# Autodesk Inventor assembly: BracoRobotico_FINAL_9999_999
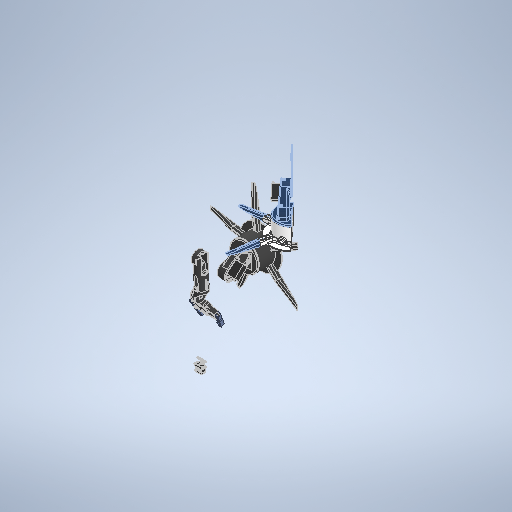
[picture p0: Inventor's stored thumbnail of the model, 512x512]
Saved by Autodesk Inventor 2025.2 (Build 292293000, 293)
## iProperties
Created: 2025-06-01
Part Number: BracoRobotico_FINAL_9999_999
Document SubType Name: Assembly
Designer: Gustavo Sousa
Author: Gustavo Sousa
## Documents named in this file (19)
- C:\Users\lucas\OneDrive\Documentos\Documentos\Gustavo\Mozangao\Projeto Base (5140)\correcao_pecas_braco_robotico\Braço Robotico peças corrigidas\BracoRobotico_FINAL_9999_999.iam
- C:\Users\lucas\OneDrive\Documentos\Documentos\Gustavo\Mozangao\Projeto Base (5140)\correcao_pecas_braco_robotico\Braço Robotico peças corrigidas\BracoRobotico_0004_001.ipt
- C:\Users\lucas\OneDrive\Documentos\Documentos\Gustavo\Mozangao\Projeto Base (5140)\correcao_pecas_braco_robotico\Braço Robotico peças corrigidas\BracoRobotico_0005_001.ipt
- C:\Users\lucas\OneDrive\Documentos\Documentos\Gustavo\Mozangao\Projeto Base (5140)\correcao_pecas_braco_robotico\Braço Robotico peças corrigidas\BracoRobotico_0002_002.ipt
- C:\Users\lucas\OneDrive\Documentos\Documentos\Gustavo\Mozangao\Projeto Base (5140)\correcao_pecas_braco_robotico\Braço Robotico peças corrigidas\BracoRobotico_0003_002.ipt
- C:\Users\lucas\OneDrive\Documentos\Documentos\Gustavo\Mozangao\Projeto Base (5140)\correcao_pecas_braco_robotico\Braço Robotico peças corrigidas\BracoRobotico_0006_001.ipt
- C:\Users\lucas\OneDrive\Documentos\Documentos\Gustavo\Mozangao\Projeto Base (5140)\correcao_pecas_braco_robotico\Braço Robotico peças corrigidas\BracoRobotico_0007_001.ipt
- C:\Users\lucas\OneDrive\Documentos\Documentos\Gustavo\Mozangao\Projeto Base (5140)\correcao_pecas_braco_robotico\Braço Robotico peças corrigidas\BracoRobotico_0008_001.ipt
- C:\Users\lucas\OneDrive\Documentos\Documentos\Gustavo\Mozangao\Projeto Base (5140)\correcao_pecas_braco_robotico\Braço Robotico peças corrigidas\Engrenagem2_0001_001.ipt
- C:\Users\lucas\OneDrive\Documentos\Documentos\Gustavo\Mozangao\Projeto Base (5140)\correcao_pecas_braco_robotico\Braço Robotico peças corrigidas\Pinza_0002_001.ipt
- C:\Users\lucas\OneDrive\Documentos\Documentos\Gustavo\Mozangao\Projeto Base (5140)\correcao_pecas_braco_robotico\Braço Robotico peças corrigidas\Barra1_0001_001.ipt
- C:\Users\lucas\OneDrive\Documentos\Documentos\Gustavo\Mozangao\Projeto Base (5140)\correcao_pecas_braco_robotico\Braço Robotico peças corrigidas\Pinza_0002_001_MIR.ipt
- C:\Users\lucas\OneDrive\Documentos\Documentos\Gustavo\Mozangao\Projeto Base (5140)\correcao_pecas_braco_robotico\Braço Robotico peças corrigidas\Engrenagem2_0001_001_MIR.ipt
- C:\Users\lucas\OneDrive\Documentos\Documentos\Gustavo\Mozangao\Projeto Base (5140)\correcao_pecas_braco_robotico\Braço Robotico peças corrigidas\Tapa_garra_0001_001.ipt
- C:\Users\lucas\OneDrive\Documentos\Documentos\Gustavo\Mozangao\Projeto Base (5140)\correcao_pecas_braco_robotico\Braço Robotico peças corrigidas\tower-pro-mg90s-micro-servo-2.snapshot.3\Tower Pro MG90S Micro se.ipt
- C:\Users\lucas\OneDrive\Documentos\Documentos\Gustavo\Mozangao\Projeto Base (5140)\correcao_pecas_braco_robotico\Braço Robotico peças corrigidas\tower-pro-mg90s-micro-servo-2.snapshot.3\Bidirectional shoulder\B.ipt
- C:\Users\lucas\OneDrive\Documentos\Documentos\Gustavo\Mozangao\Projeto Base (5140)\correcao_pecas_braco_robotico\Braço Robotico peças corrigidas\mg995-servo-motor-1.snapshot.1\MG995 Servo Motor\servo Assem\serv.ipt
- C:\Users\lucas\OneDrive\Documentos\Documentos\Gustavo\Mozangao\Projeto Base (5140)\correcao_pecas_braco_robotico\Brazo Robótivo 2023 v144\Brazo Robótivo 2023 v144\Brazo Robótivo 2023 v144.iam
- C:\Users\lucas\OneDrive\Documentos\Documentos\Gustavo\Mozangao\Projeto Base (5140)\correcao_pecas_braco_robotico\Braço Robotico peças corrigidas\mg995-servo-motor-1.snapshot.1\MG995 Servo Motor\servo strong jun.ipt
## Components (24 placed, 18 different names)
1. BracoRobotico_0004_001:1 — Coincidente:1, Coincidente:2, Alinhado:1, Inserir:1, Coincidente:3, Coincidente:4, Coincidente:5, Coincidente:6, Coincidente:7, Coincidente:8, Coincidente:9, Coincidente:10, Coincidente:11, Coincidente:12, Coincidente:13, Coincidente:14, Coincidente:15, Coincidente:16, Coincidente:17, Coincidente:44, Coincidente:45, Coincidente:46
2. BracoRobotico_0005_001:1 — Inserir:1, Inserir:2, Coincidente:47, Coincidente:48, Coincidente:49
3. BracoRobotico_0002_002:1 — Inserir:2, Inserir:3
4. BracoRobotico_0003_002:1 — Coincidente:6, Coincidente:7, Coincidente:8
5. BracoRobotico_0003_002:2 — Coincidente:12, Coincidente:13, Coincidente:14
6. BracoRobotico_0003_002:3 — Coincidente:9, Coincidente:10, Coincidente:11
7. BracoRobotico_0003_002:4 — Coincidente:15, Coincidente:16, Coincidente:17
8. BracoRobotico_0003_002:5 — Coincidente:3, Coincidente:4, Coincidente:5
9. BracoRobotico_0006_001:1 — Inserir:3, Inserir:4
10. BracoRobotico_0007_001:1 — Coincidente:26, Coincidente:27, Inserir:4
11. BracoRobotico_0008_001:1 — Coincidente:23, Coincidente:24, Coincidente:25, Coincidente:26, Coincidente:27, Coincidente:28, Coincidente:29, Coincidente:30, Coincidente:31, Coincidente:32, Coincidente:33, Coincidente:34, Coincidente:35, Coincidente:42, Coincidente:43
12. Engrenagem2_0001_001:1 — Coincidente:28, Coincidente:29, Coincidente:39, Coincidente:40, Coincidente:43
13. Engrenagem2_0001_001_MIR:1 — Coincidente:30, Coincidente:31, Coincidente:36, Coincidente:37, Coincidente:42
14. Pinza_0002_001_MIR:1 — Coincidente:39, Coincidente:40, Coincidente:41
15. Pinza_0002_001:1 — Coincidente:36, Coincidente:37, Coincidente:38
16. Barra1_0001_001:1 — Coincidente:32, Coincidente:33, Coincidente:41
17. Barra1_0001_001:2 — Coincidente:34, Coincidente:35, Coincidente:38
18. Tapa_garra_0001_001:1 — Coincidente:23, Coincidente:24, Coincidente:25
19. Tower Pro MG90S Micro se:1
20. B:1
21. serv:1 — Coincidente:44, Coincidente:45, Coincidente:46
22. serv:2 — Coincidente:47, Coincidente:48, Coincidente:49
23. Brazo Robótivo 2023 v144:1 [sub-assembly] — Coincidente:50, Coincidente:51, Coincidente:52
24. servo strong jun:1 — Coincidente:50, Coincidente:51, Coincidente:52
## Relationships (52: Mate 47, Insert 4, Flush 1)
- Coincidente:1 [Mate]: BracoRobotico_0004_001:1
- Coincidente:2 [Mate]: BracoRobotico_0004_001:1
- Alinhado:1 [Flush]: BracoRobotico_0004_001:1
- Inserir:1: BracoRobotico_0004_001:1 ↔ BracoRobotico_0005_001:1
- Inserir:2: BracoRobotico_0005_001:1 ↔ BracoRobotico_0002_002:1
- Coincidente:3 [Mate]: BracoRobotico_0004_001:1 ↔ BracoRobotico_0003_002:5
- Coincidente:4 [Mate]: BracoRobotico_0004_001:1 ↔ BracoRobotico_0003_002:5
- Coincidente:5 [Mate]: BracoRobotico_0004_001:1 ↔ BracoRobotico_0003_002:5
- Coincidente:6 [Mate]: BracoRobotico_0004_001:1 ↔ BracoRobotico_0003_002:1
- Coincidente:7 [Mate]: BracoRobotico_0004_001:1 ↔ BracoRobotico_0003_002:1
- Coincidente:8 [Mate]: BracoRobotico_0004_001:1 ↔ BracoRobotico_0003_002:1
- Coincidente:9 [Mate]: BracoRobotico_0004_001:1 ↔ BracoRobotico_0003_002:3
- Coincidente:10 [Mate]: BracoRobotico_0004_001:1 ↔ BracoRobotico_0003_002:3
- Coincidente:11 [Mate]: BracoRobotico_0004_001:1 ↔ BracoRobotico_0003_002:3
- Coincidente:12 [Mate]: BracoRobotico_0004_001:1 ↔ BracoRobotico_0003_002:2
- Coincidente:13 [Mate]: BracoRobotico_0004_001:1 ↔ BracoRobotico_0003_002:2
- Coincidente:14 [Mate]: BracoRobotico_0004_001:1 ↔ BracoRobotico_0003_002:2
- Coincidente:15 [Mate]: BracoRobotico_0004_001:1 ↔ BracoRobotico_0003_002:4
- Coincidente:16 [Mate]: BracoRobotico_0004_001:1 ↔ BracoRobotico_0003_002:4
- Coincidente:17 [Mate]: BracoRobotico_0004_001:1 ↔ BracoRobotico_0003_002:4
- Inserir:3: BracoRobotico_0002_002:1 ↔ BracoRobotico_0006_001:1
- Coincidente:23 [Mate]: BracoRobotico_0008_001:1 ↔ Tapa_garra_0001_001:1
- Coincidente:24 [Mate]: BracoRobotico_0008_001:1 ↔ Tapa_garra_0001_001:1
- Coincidente:25 [Mate] (0.165 mm): BracoRobotico_0008_001:1 ↔ Tapa_garra_0001_001:1
- Coincidente:26 [Mate]: BracoRobotico_0007_001:1 ↔ BracoRobotico_0008_001:1
- Coincidente:27 [Mate]: BracoRobotico_0007_001:1 ↔ BracoRobotico_0008_001:1
- Coincidente:28 [Mate]: BracoRobotico_0008_001:1 ↔ Engrenagem2_0001_001:1
- Coincidente:29 [Mate]: BracoRobotico_0008_001:1 ↔ Engrenagem2_0001_001:1
- Coincidente:30 [Mate]: BracoRobotico_0008_001:1 ↔ Engrenagem2_0001_001_MIR:1
- Coincidente:31 [Mate]: BracoRobotico_0008_001:1 ↔ Engrenagem2_0001_001_MIR:1
- Coincidente:32 [Mate] (0.8 mm): BracoRobotico_0008_001:1 ↔ Barra1_0001_001:1
- Coincidente:33 [Mate]: BracoRobotico_0008_001:1 ↔ Barra1_0001_001:1
- Coincidente:34 [Mate] (0.8 mm): BracoRobotico_0008_001:1 ↔ Barra1_0001_001:2
- Coincidente:35 [Mate]: BracoRobotico_0008_001:1 ↔ Barra1_0001_001:2
- Coincidente:36 [Mate] (0.35 mm): Engrenagem2_0001_001_MIR:1 ↔ Pinza_0002_001:1
- Coincidente:37 [Mate]: Engrenagem2_0001_001_MIR:1 ↔ Pinza_0002_001:1
- Coincidente:38 [Mate]: Pinza_0002_001:1 ↔ Barra1_0001_001:2
- Coincidente:39 [Mate] (0.35 mm): Engrenagem2_0001_001:1 ↔ Pinza_0002_001_MIR:1
- Coincidente:40 [Mate]: Engrenagem2_0001_001:1 ↔ Pinza_0002_001_MIR:1
- Coincidente:41 [Mate]: Pinza_0002_001_MIR:1 ↔ Barra1_0001_001:1
- Inserir:4: BracoRobotico_0006_001:1 ↔ BracoRobotico_0007_001:1
- Coincidente:42 [Mate] (5.296 mm): BracoRobotico_0008_001:1 ↔ Engrenagem2_0001_001_MIR:1
- Coincidente:43 [Mate] (4.743 mm): BracoRobotico_0008_001:1 ↔ Engrenagem2_0001_001:1
- Coincidente:44 [Mate]: BracoRobotico_0004_001:1 ↔ serv:1
- Coincidente:45 [Mate]: BracoRobotico_0004_001:1 ↔ serv:1
- Coincidente:46 [Mate]: BracoRobotico_0004_001:1 ↔ serv:1
- Coincidente:47 [Mate]: BracoRobotico_0005_001:1 ↔ serv:2
- Coincidente:48 [Mate]: BracoRobotico_0005_001:1 ↔ serv:2
- Coincidente:49 [Mate]: BracoRobotico_0005_001:1 ↔ serv:2
- Coincidente:50 [Mate]: Brazo Robótivo 2023 v144:1 ↔ servo strong jun:1
- Coincidente:51 [Mate]: Brazo Robótivo 2023 v144:1 ↔ servo strong jun:1
- Coincidente:52 [Mate]: Brazo Robótivo 2023 v144:1 ↔ servo strong jun:1
